# Autodesk Inventor assembly: WheelEncoderBoardLarger
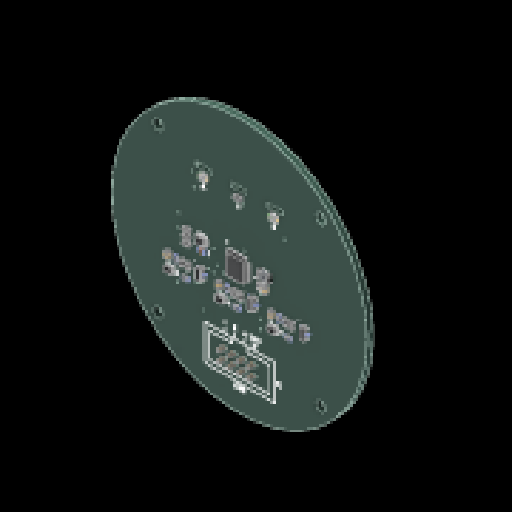
[picture p0: Inventor's stored thumbnail of the model, 512x512]
Saved by Autodesk Inventor 2025.2 (Build 292293000, 293)
## iProperties
Company: Kicad
Created: 2026-02-08
Part Number: WheelEncoderBoardLarger
Description: KiCad electronic assembly
Document SubType Name: Assembly
Designer: valer
Authority: Unknown
Sending System: KiCad to STEP converter
Preprocessor: Open CASCADE STEP processor 7.8
Title: LegEncoderBoardLarger.step
Author: Pcbnew
## Documents named in this file (21)
- C:\Users\valer\Desktop\str1ker\cad\external\WheelEncoder\WheelEncoderBoard.iam
- C:\Users\valer\Desktop\str1ker\cad\external\WheelEncoder\CC0603JRX7R7BB105.ipt
- C:\Users\valer\Desktop\str1ker\cad\external\WheelEncoder\RC0603FR-0722RL.ipt
- C:\Users\valer\Desktop\str1ker\cad\external\WheelEncoder\RCG06031K00FKEA.ipt
- C:\Users\valer\Desktop\str1ker\cad\external\WheelEncoder\RC0603FR-07150RL.ipt
- C:\Users\valer\Desktop\str1ker\cad\external\WheelEncoder\RC0603FR-07470KL.ipt
- C:\Users\valer\Desktop\str1ker\cad\external\WheelEncoder\BAT54WS-7-F.ipt
- C:\Users\valer\Desktop\str1ker\cad\external\WheelEncoder\885012206089.iam
- C:\Users\valer\Desktop\str1ker\cad\external\WheelEncoder\TSSOP-14_AMS.ipt
- C:\Users\valer\Desktop\str1ker\cad\external\WheelEncoder\GRM188R71H104KA93J.ipt
- C:\Users\valer\Desktop\str1ker\cad\external\WheelEncoder\885342208002.iam
- C:\Users\valer\Desktop\str1ker\cad\external\WheelEncoder\IDC-Header_2x04_P2.54mm_Vertical.ipt
- C:\Users\valer\Desktop\str1ker\cad\external\WheelEncoder\SN74LVC3G17DCUR.iam
- C:\Users\valer\Desktop\str1ker\cad\external\WheelEncoder\MMBT3904LT1G.ipt
- C:\Users\valer\Desktop\str1ker\cad\external\WheelEncoder\150080BS75000.iam
- C:\Users\valer\Desktop\str1ker\cad\external\WheelEncoder\RC0603FR-07150RL_1.ipt
- C:\Users\valer\Desktop\str1ker\cad\external\WheelEncoder\CRCW0603100KFKEA.ipt
- C:\Users\valer\Desktop\str1ker\cad\external\WheelEncoder\RC0603FR-0747KL.ipt
- C:\Users\valer\Desktop\str1ker\cad\external\WheelEncoder\LegEncoderBoard_silkscreen.ipt
- C:\Users\valer\Desktop\str1ker\cad\external\WheelEncoder\LegEncoderBoard_silkscreen_1.ipt
- C:\Users\valer\Desktop\str1ker\cad\external\WheelEncoder\LegEncoderBoard_PCB.ipt
## Components (37 placed, 37 different names)
1. 1
2. 2
3. 3
4. 4
5. 5
6. 6
7. 7
8. 8
9. 12 [sub-assembly]
10. 13
11. 14
12. 15
13. 19 [sub-assembly]
14. 20 — Flush:1, Mate:3, Mate:1
15. 30 [sub-assembly]
16. 31
17. 38 [sub-assembly]
18. 39
19. 40
20. 41
21. 42
22. 43
23. 44
24. 45
25. 46
26. 47 [sub-assembly]
27. 48
28. 49
29. 50
30. 51
31. 52
32. 53
33. 54
34. 55
35. 56
36. 57
37. 58 — Mate:1
## Relationships (3: Mate 2, Flush 1)
- Flush:1 (-17.093 mm): 20
- Mate:3 (-9.125 mm): 20
- Mate:1: 20 ↔ 58
